# Autodesk Inventor assembly: КВ33.044.900 - Каретка оси X
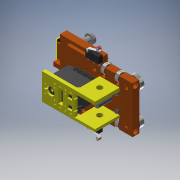
[picture p0: Inventor's stored thumbnail of the model, 180x180]
Saved by Autodesk Inventor 2019 (Build 230136000, 136)
## iProperties
Created: 2019-08-08
Part Number: КВ33.044.900 - Каретка оси X
Material: Типовые
Document SubType Name: Assembly
Designer: user
Author: user
## Documents named in this file (15)
- C:\Users\user\Documents\Kvantoriada2019\optimal_gripper\hardware\КВ33.044.300 - Каретка оси X.iam
- C:\Users\user\Documents\Kvantoriada2019\optimal_gripper\hardware\КВ33.044.301 - Щека каретки X.ipt
- C:\Users\user\Documents\Kvantoriada2019\optimal_gripper\hardware\Стандартные изделия\Подшипник 624Z.ipt
- C:\Users\user\Documents\Kvantoriada2019\optimal_gripper\hardware\Стандартные изделия\Подшипник 626Z.ipt
- C:\Users\user\Documents\Kvantoriada2019\optimal_gripper\hardware\Стандартные изделия\Винт М8х25 с потайной головкой.ipt
- C:\Users\user\Documents\Kvantoriada2019\optimal_gripper\hardware\Стандартные изделия\Винт М5х10 с потайной головкой.ipt
- C:\Users\user\Documents\Kvantoriada2019\optimal_gripper\hardware\Стандартные изделия\Сервомотор Dynamixel AX-12A\ax-12a.iam
- C:\Users\user\Documents\Kvantoriada2019\optimal_gripper\hardware\КВ33.044.304 -Проставка 6 мм.ipt
- C:\Users\user\Documents\Kvantoriada2019\optimal_gripper\hardware\КВ33.044.404 - Колесо энкодера.ipt
- C:\Users\user\Documents\Kvantoriada2019\optimal_gripper\hardware\Стандартные изделия\Шкив большой Makeblock.ipt
- C:\Users\user\Documents\Kvantoriada2019\optimal_gripper\hardware\КВ33.044.405 -  Боковина шкива.ipt
- C:\Users\user\Documents\Kvantoriada2019\optimal_gripper\hardware\Стандартные изделия\Датчик оптический (стандартный).ipt
- C:\Users\user\Documents\Kvantoriada2019\optimal_gripper\hardware\Стандартные изделия\Концевик механический\Концевик механический.ipt
- C:\Users\user\Documents\Kvantoriada2019\optimal_gripper\hardware\КВ33.044.800 - Шкив плоский Makeblock сборка.iam
- C:\Users\user\Documents\Kvantoriada2019\optimal_gripper\hardware\КВ33.044.305 - Крепеж ремня оси Y.ipt
## Components (25 placed, 14 different names)
1. КВ33.044.301 - Щека каретки X:1 — Совмещение:1, Совмещение:2, Совмещение:3, Совмещение:4, Совмещение:5, Совмещение:6, Совмещение:7, Совмещение:8, Совмещение:9, Совмещение:10, Совмещение:11, Совмещение:12, Совмещение:13, Совмещение:14, Совмещение:15, Совмещение:16, Совмещение:17, Заподлицо:1, Совмещение:18, Заподлицо:2, Совмещение:19, Заподлицо:3, Совмещение:20, Заподлицо:4, Совмещение:21, Заподлицо:5, Совмещение:22, Совмещение:23, Совмещение:24, Совмещение:39, Совмещение:40, Заподлицо:6, Совмещение:41, Совмещение:42, Совмещение:43, Совмещение:44, Совмещение:45, Совмещение:46, Касательность:1, Касательность:2, Совмещение:47, Совмещение:48
2. Подшипник 624Z:1 — Совмещение:1, Совмещение:2
3. Подшипник 624Z:2 — Совмещение:3, Совмещение:4
4. Подшипник 624Z:3 — Совмещение:7, Совмещение:8
5. Подшипник 624Z:4 — Совмещение:5, Совмещение:6
6. Подшипник 626Z:1 — Совмещение:9, Совмещение:10
7. Подшипник 626Z:2 — Совмещение:13, Совмещение:14
8. Подшипник 626Z:3 — Совмещение:11, Совмещение:12
9. Подшипник 626Z:4 — Совмещение:15, Совмещение:16
10. Винт М8х25 с потайной головкой:1 — Совмещение:17, Заподлицо:1
11. Винт М5х10 с потайной головкой:1 — Совмещение:19, Заподлицо:3
12. Винт М5х10 с потайной головкой:2 — Совмещение:21, Заподлицо:5
13. Винт М5х10 с потайной головкой:3 — Совмещение:18, Заподлицо:2
14. Винт М5х10 с потайной головкой:4 — Совмещение:20, Заподлицо:4
15. ax-12a:1 [sub-assembly] — Совмещение:22, Совмещение:23, Совмещение:24, Совмещение:25, Совмещение:26, Совмещение:49, Совмещение:50, Совмещение:51
16. КВ33.044.304 -Проставка 6 мм:1 — Совмещение:25, Совмещение:26, Совмещение:27, Совмещение:28, Совмещение:29
17. КВ33.044.404 - Колесо энкодера:1 — Совмещение:27, Совмещение:28, Совмещение:29, Совмещение:30, Совмещение:31, Совмещение:32
18. Шкив большой Makeblock:1 — Совмещение:30, Совмещение:31, Совмещение:32, Совмещение:33, Совмещение:34, Совмещение:35
19. КВ33.044.405 -  Боковина шкива:1 — Совмещение:33, Совмещение:34, Совмещение:35
20. Датчик оптический (стандартный):1 — Совмещение:39, Совмещение:40, Заподлицо:6
21. Концевик механический:1 — Совмещение:41, Совмещение:42, Совмещение:43
22. Концевик механический:2 — Совмещение:44, Совмещение:45, Совмещение:46
23. КВ33.044.800 - Шкив плоский Makeblock сборка:1 [sub-assembly] — Касательность:1, Совмещение:48
24. КВ33.044.800 - Шкив плоский Makeblock сборка:2 [sub-assembly] — Касательность:2, Совмещение:47
25. КВ33.044.305 - Крепеж ремня оси Y:1 — Совмещение:49, Совмещение:50, Совмещение:51
## Relationships (56: Mate 48, Flush 6, Tangent 2)
- Совмещение:1 [Mate]: КВ33.044.301 - Щека каретки X:1 ↔ Подшипник 624Z:1
- Совмещение:2 [Mate] (0.5 mm): КВ33.044.301 - Щека каретки X:1 ↔ Подшипник 624Z:1
- Совмещение:3 [Mate]: КВ33.044.301 - Щека каретки X:1 ↔ Подшипник 624Z:2
- Совмещение:4 [Mate] (0.5 mm): КВ33.044.301 - Щека каретки X:1 ↔ Подшипник 624Z:2
- Совмещение:5 [Mate] (0.5 mm): КВ33.044.301 - Щека каретки X:1 ↔ Подшипник 624Z:4
- Совмещение:6 [Mate]: КВ33.044.301 - Щека каретки X:1 ↔ Подшипник 624Z:4
- Совмещение:7 [Mate]: КВ33.044.301 - Щека каретки X:1 ↔ Подшипник 624Z:3
- Совмещение:8 [Mate] (0.5 mm): КВ33.044.301 - Щека каретки X:1 ↔ Подшипник 624Z:3
- Совмещение:9 [Mate]: КВ33.044.301 - Щека каретки X:1 ↔ Подшипник 626Z:1
- Совмещение:10 [Mate] (2 mm): КВ33.044.301 - Щека каретки X:1 ↔ Подшипник 626Z:1
- Совмещение:11 [Mate]: КВ33.044.301 - Щека каретки X:1 ↔ Подшипник 626Z:3
- Совмещение:12 [Mate] (2 mm): КВ33.044.301 - Щека каретки X:1 ↔ Подшипник 626Z:3
- Совмещение:13 [Mate]: КВ33.044.301 - Щека каретки X:1 ↔ Подшипник 626Z:2
- Совмещение:14 [Mate] (2 mm): КВ33.044.301 - Щека каретки X:1 ↔ Подшипник 626Z:2
- Совмещение:15 [Mate]: КВ33.044.301 - Щека каретки X:1 ↔ Подшипник 626Z:4
- Совмещение:16 [Mate] (2 mm): КВ33.044.301 - Щека каретки X:1 ↔ Подшипник 626Z:4
- Совмещение:17 [Mate]: КВ33.044.301 - Щека каретки X:1 ↔ Винт М8х25 с потайной головкой:1
- Заподлицо:1 [Flush] (2 mm): КВ33.044.301 - Щека каретки X:1 ↔ Винт М8х25 с потайной головкой:1
- Совмещение:18 [Mate]: КВ33.044.301 - Щека каретки X:1 ↔ Винт М5х10 с потайной головкой:3
- Заподлицо:2 [Flush] (1 mm): КВ33.044.301 - Щека каретки X:1 ↔ Винт М5х10 с потайной головкой:3
- Совмещение:19 [Mate]: КВ33.044.301 - Щека каретки X:1 ↔ Винт М5х10 с потайной головкой:1
- Заподлицо:3 [Flush] (1 mm): КВ33.044.301 - Щека каретки X:1 ↔ Винт М5х10 с потайной головкой:1
- Совмещение:20 [Mate]: КВ33.044.301 - Щека каретки X:1 ↔ Винт М5х10 с потайной головкой:4
- Заподлицо:4 [Flush] (1 mm): КВ33.044.301 - Щека каретки X:1 ↔ Винт М5х10 с потайной головкой:4
- Совмещение:21 [Mate]: КВ33.044.301 - Щека каретки X:1 ↔ Винт М5х10 с потайной головкой:2
- Заподлицо:5 [Flush] (1 mm): КВ33.044.301 - Щека каретки X:1 ↔ Винт М5х10 с потайной головкой:2
- Совмещение:22 [Mate]: КВ33.044.301 - Щека каретки X:1 ↔ ax-12a:1
- Совмещение:23 [Mate]: КВ33.044.301 - Щека каретки X:1 ↔ ax-12a:1
- Совмещение:24 [Mate]: КВ33.044.301 - Щека каретки X:1 ↔ ax-12a:1
- Совмещение:25 [Mate]: ax-12a:1 ↔ КВ33.044.304 -Проставка 6 мм:1
- Совмещение:26 [Mate]: ax-12a:1 ↔ КВ33.044.304 -Проставка 6 мм:1
- Совмещение:27 [Mate]: КВ33.044.304 -Проставка 6 мм:1 ↔ КВ33.044.404 - Колесо энкодера:1
- Совмещение:28 [Mate]: КВ33.044.304 -Проставка 6 мм:1 ↔ КВ33.044.404 - Колесо энкодера:1
- Совмещение:29 [Mate]: КВ33.044.304 -Проставка 6 мм:1 ↔ КВ33.044.404 - Колесо энкодера:1
- Совмещение:30 [Mate]: КВ33.044.404 - Колесо энкодера:1 ↔ Шкив большой Makeblock:1
- Совмещение:31 [Mate]: КВ33.044.404 - Колесо энкодера:1 ↔ Шкив большой Makeblock:1
- Совмещение:32 [Mate]: КВ33.044.404 - Колесо энкодера:1 ↔ Шкив большой Makeblock:1
- Совмещение:33 [Mate]: Шкив большой Makeblock:1 ↔ КВ33.044.405 -  Боковина шкива:1
- Совмещение:34 [Mate]: Шкив большой Makeblock:1 ↔ КВ33.044.405 -  Боковина шкива:1
- Совмещение:35 [Mate]: Шкив большой Makeblock:1 ↔ КВ33.044.405 -  Боковина шкива:1
- Совмещение:39 [Mate] (10 mm): КВ33.044.301 - Щека каретки X:1 ↔ Датчик оптический (стандартный):1
- Совмещение:40 [Mate] (-4.7 mm): КВ33.044.301 - Щека каретки X:1 ↔ Датчик оптический (стандартный):1
- Заподлицо:6 [Flush] (15 mm): КВ33.044.301 - Щека каретки X:1 ↔ Датчик оптический (стандартный):1
- Совмещение:41 [Mate]: КВ33.044.301 - Щека каретки X:1 ↔ Концевик механический:1
- Совмещение:42 [Mate]: КВ33.044.301 - Щека каретки X:1 ↔ Концевик механический:1
- Совмещение:43 [Mate]: КВ33.044.301 - Щека каретки X:1 ↔ Концевик механический:1
- Совмещение:44 [Mate]: КВ33.044.301 - Щека каретки X:1 ↔ Концевик механический:2
- Совмещение:45 [Mate]: КВ33.044.301 - Щека каретки X:1 ↔ Концевик механический:2
- Совмещение:46 [Mate]: КВ33.044.301 - Щека каретки X:1 ↔ Концевик механический:2
- Касательность:1 [Tangent]: КВ33.044.301 - Щека каретки X:1 ↔ КВ33.044.800 - Шкив плоский Makeblock сборка:1
- Касательность:2 [Tangent]: КВ33.044.301 - Щека каретки X:1 ↔ КВ33.044.800 - Шкив плоский Makeblock сборка:2
- Совмещение:47 [Mate]: КВ33.044.301 - Щека каретки X:1 ↔ КВ33.044.800 - Шкив плоский Makeblock сборка:2
- Совмещение:48 [Mate]: КВ33.044.301 - Щека каретки X:1 ↔ КВ33.044.800 - Шкив плоский Makeblock сборка:1
- Совмещение:49 [Mate]: ax-12a:1 ↔ КВ33.044.305 - Крепеж ремня оси Y:1
- Совмещение:50 [Mate]: ax-12a:1 ↔ КВ33.044.305 - Крепеж ремня оси Y:1
- Совмещение:51 [Mate]: ax-12a:1 ↔ КВ33.044.305 - Крепеж ремня оси Y:1
